# Autodesk Inventor assembly: BC-100000-Sup
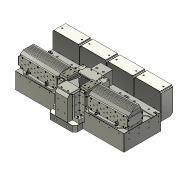
[picture p0: Inventor's stored thumbnail of the model, 180x180]
Saved by Autodesk Inventor 2016 (Build 200138000, 138)
## iProperties
Created: 2015-09-16
Part Number: BC-100000-Sup
Document SubType Name: Assembly
Designer: Reinaldo.Basílio
Mass: 567958 g
Surface Area: 49385.8 cm^2
Volume: 75452.4 cm^3
Density: 7.52737 g/cm^3
Author: Reinaldo.Basílio
## Documents named in this file (40)
- D:\ARQ\Basilio\LNLS-2\Anel\Dipolos\BC-3T\Dipolo 3T e 1T\Prototipo 1\Projeto Mecanico\BC-100000-Sup.iam
- D:\ARQ\Basilio\LNLS-2\Anel\Dipolos\BC-3T\Dipolo 3T e 1T\Prototipo 1\Projeto Mecanico\BC-100004.iam
- D:\ARQ\Basilio\LNLS-2\Anel\Dipolos\BC-3T\Dipolo 3T e 1T\Prototipo 1\Projeto Mecanico\BC-10005.ipt
- D:\ARQ\Basilio\LNLS-2\Anel\Dipolos\BC-3T\Dipolo 3T e 1T\Prototipo 1\Projeto Mecanico\BC-100005.iam
- D:\ARQ\Basilio\LNLS-2\Anel\Dipolos\BC-3T\Dipolo 3T e 1T\Prototipo 1\Projeto Mecanico\BC-10008.ipt
- D:\ARQ\Basilio\LNLS-2\Anel\Dipolos\BC-3T\Dipolo 3T e 1T\Prototipo 1\Projeto Mecanico\BC-10007.ipt
- D:\ARQ\Basilio\LNLS-2\Anel\Dipolos\BC-3T\Dipolo 3T e 1T\Prototipo 1\Projeto Mecanico\BC-10001.ipt
- D:\ARQ\Basilio\LNLS-2\Anel\Dipolos\BC-3T\Dipolo 3T e 1T\Prototipo 1\Projeto Mecanico\BC-10019-A.ipt
- D:\ARQ\Basilio\LNLS-2\Anel\Dipolos\BC-3T\Dipolo 3T e 1T\Prototipo 1\Projeto Mecanico\BC-10002.ipt
- D:\ARQ\Basilio\LNLS-2\Anel\Dipolos\BC-3T\Dipolo 3T e 1T\Prototipo 1\Projeto Mecanico\BC-10011.ipt
- D:\ARQ\Basilio\LNLS-2\Anel\Dipolos\BC-3T\Dipolo 3T e 1T\Prototipo 1\Projeto Mecanico\BC-10012.ipt
- D:\ARQ\Basilio\LNLS-2\Anel\Dipolos\BC-3T\Dipolo 3T e 1T\Prototipo 1\Projeto Mecanico\BC-10013.ipt
- D:\ARQ\Basilio\LNLS-2\Anel\Dipolos\BC-3T\Dipolo 3T e 1T\Prototipo 1\Projeto Mecanico\BC-10014.ipt
- D:\ARQ\Basilio\LNLS-2\Anel\Dipolos\BC-3T\Dipolo 3T e 1T\Prototipo 1\Projeto Mecanico\BC-10019-B.ipt
- D:\ARQ\Basilio\LNLS-2\Anel\Dipolos\BC-3T\Dipolo 3T e 1T\Prototipo 1\Projeto Mecanico\BC-10015.ipt
- D:\ARQ\Basilio\LNLS-2\Anel\Dipolos\BC-3T\Dipolo 3T e 1T\Prototipo 1\Projeto Mecanico\BC-10016.ipt
- D:\ARQ\Basilio\LNLS-2\Anel\Dipolos\BC-3T\Dipolo 3T e 1T\Prototipo 1\Projeto Mecanico\BC-10009.ipt
- D:\ARQ\Basilio\LNLS-2\Anel\Dipolos\BC-3T\Dipolo 3T e 1T\Prototipo 1\Projeto Mecanico\BC-100001-A-Sup.iam
- D:\ARQ\Basilio\LNLS-2\Anel\Dipolos\BC-3T\Dipolo 3T e 1T\Prototipo 1\Projeto Mecanico\BC-100001-B-Sup.iam
- D:\ARQ\Basilio\LNLS-2\Anel\Dipolos\BC-3T\Dipolo 3T e 1T\Prototipo 1\Projeto Mecanico\BC-10021.ipt
- D:\ARQ\Basilio\LNLS-2\Anel\Dipolos\BC-3T\Dipolo 3T e 1T\Prototipo 1\Projeto Mecanico\BC-10022.ipt
- D:\ARQ\Basilio\LNLS-2\Anel\Dipolos\BC-3T\Dipolo 3T e 1T\Prototipo 1\Projeto Mecanico\BC-10025.ipt
- D:\ARQ\Basilio\LNLS-2\Anel\Dipolos\BC-3T\Dipolo 3T e 1T\Prototipo 1\Projeto Mecanico\Parafusos\DIN 912 - M12x65.ipt
- D:\ARQ\Basilio\LNLS-2\Anel\Dipolos\BC-3T\Dipolo 3T e 1T\Prototipo 1\Projeto Mecanico\BC-10020.ipt
- D:\ARQ\Basilio\LNLS-2\Anel\Dipolos\BC-3T\Dipolo 3T e 1T\Prototipo 1\Projeto Mecanico\Parafusos\DIN 912 - M8x30.ipt
- D:\ARQ\Basilio\LNLS-2\Anel\Dipolos\BC-3T\Dipolo 3T e 1T\Prototipo 1\Projeto Mecanico\Parafusos\DIN 912 - M8x80.ipt
- D:\ARQ\Basilio\LNLS-2\Anel\Dipolos\BC-3T\Dipolo 3T e 1T\Prototipo 1\Projeto Mecanico\Parafusos\DIN 912 - M10x50.ipt
- D:\ARQ\Basilio\LNLS-2\Anel\Dipolos\BC-3T\Dipolo 3T e 1T\Prototipo 1\Projeto Mecanico\Parafusos\DIN 912 - M4x12.ipt
- D:\ARQ\Basilio\LNLS-2\Anel\Dipolos\BC-3T\Dipolo 3T e 1T\Prototipo 1\Projeto Mecanico\Parafusos\DIN 912 - M5x16.ipt
- D:\ARQ\Basilio\LNLS-2\Anel\Dipolos\BC-3T\Dipolo 3T e 1T\Prototipo 1\Projeto Mecanico\BC-10023.ipt
- D:\ARQ\Basilio\LNLS-2\Anel\Dipolos\BC-3T\Dipolo 3T e 1T\Prototipo 1\Projeto Mecanico\Parafusos\DIN 7991 - M5x12.ipt
- D:\ARQ\Basilio\LNLS-2\Anel\Dipolos\BC-3T\Dipolo 3T e 1T\Prototipo 1\Projeto Mecanico\Parafusos\DIN 125 - A 10,5.ipt
- D:\ARQ\Basilio\LNLS-2\Anel\Dipolos\BC-3T\Dipolo 3T e 1T\Prototipo 1\Projeto Mecanico\Parafusos\DIN 912 - M10x40.ipt
- D:\ARQ\Basilio\LNLS-2\Anel\Dipolos\BC-3T\Dipolo 3T e 1T\Prototipo 1\Projeto Mecanico\Parafusos\DIN 912 - M8x20.ipt
- D:\ARQ\Basilio\LNLS-2\Anel\Dipolos\BC-3T\Dipolo 3T e 1T\Prototipo 1\Projeto Mecanico\Parafusos\DIN 912 - M8x40.ipt
- D:\ARQ\Basilio\LNLS-2\Anel\Dipolos\BC-3T\Dipolo 3T e 1T\Prototipo 1\Projeto Mecanico\Parafusos\DIN 933 - M4x14.ipt
- D:\ARQ\Basilio\LNLS-2\Anel\Dipolos\BC-3T\Dipolo 3T e 1T\Prototipo 1\Projeto Mecanico\Parafusos\DIN 912 - M4x18.ipt
- D:\ARQ\Basilio\LNLS-2\Anel\Dipolos\BC-3T\Dipolo 3T e 1T\Prototipo 1\Projeto Mecanico\BC-10026.ipt
- D:\ARQ\Basilio\LNLS-2\Anel\Dipolos\BC-3T\Dipolo 3T e 1T\Prototipo 1\Projeto Mecanico\BC-10027.ipt
- D:\ARQ\Basilio\LNLS-2\Anel\Dipolos\BC-3T\Dipolo 3T e 1T\Prototipo 1\Projeto Mecanico\BC-100001\AIP\FEA\bjj5sjykh.fres
## Components (139 placed, 38 different names)
1. BC-10001:1 — Flush:41, Mate:39, Mate:48, Insert:3, Insert:6, Insert:7, Insert:8, Mate:54, Mate:55, Insert:13, Insert:15, Insert:16, Insert:22, Insert:23, Insert:24, Insert:25, Insert:26, Insert:27, Mate:57, Mate:62, Insert:30, Insert:31, Insert:36, Insert:37, Insert:38, Insert:39, Insert:40, Insert:41, Insert:42, Insert:43, Insert:44, Insert:45, Mate:67, Mate:70, Insert:61, Insert:62, Insert:71, Insert:72, Insert:73, Insert:74, Insert:75, Insert:76, Insert:77, Insert:78, Insert:167, Insert:168
2. BC-10002:1 — Flush:46, Mate:48, Insert:17, Insert:18, Insert:19, Insert:20, Insert:44, Insert:45, Flush:47, Insert:54, Insert:55, Insert:87, Insert:88
3. BC-100005:1 [sub-assembly] — Flush:28, Mate:67, Flush:47
4. BC-100004:1 [sub-assembly] — Mate:69, Flush:25, Mate:68, Mate:70
5. BC-10019-B:1 — Insert:13, Insert:14, Insert:131, Insert:132, Insert:133, Insert:134
6. BC-10019-A:2 — Mate:39, Mate:40, Mate:41, Insert:123, Insert:124, Insert:125, Insert:126
7. BC-10005:1 — Flush:25, Flush:28, Mate:22, Mate:24, Mate:28, Flush:33, Mate:29, Flush:34, Flush:41, Mate:40, Mate:41, Flush:46, Insert:14, Mate:68, Flush:48, Mate:71, Flush:49, Flush:51
8. BC-100004:2 [sub-assembly] — Mate:22, Flush:31, Flush:48
9. BC-100004:3 [sub-assembly] — Mate:24, Flush:50, Flush:51
10. BC-100005:2 [sub-assembly] — Flush:31, Flush:34, Mate:71, Flush:49, Flush:50
11. BC-10008:1 — Insert:28, Insert:29, Insert:30, Insert:31, Insert:46, Insert:47, Insert:48, Insert:49, Insert:93, Insert:94, Insert:95, Insert:96
12. BC-10007:1 — Insert:28, Insert:29
13. BC-100001-A-Sup:1 [sub-assembly] — Insert:3, Tangent:2, Mate:54
14. BC-100001-B-Sup:1 [sub-assembly] — Insert:6, Tangent:1, Mate:55
15. BC-10011:1 — Insert:8, Tangent:1, Insert:158
16. BC-10011:2 — Insert:7, Tangent:2, Insert:157
17. BC-10012:1 — Insert:15, Insert:16, Insert:149, Insert:150
18. BC-10014:1 — Insert:17, Insert:18, Insert:144, Insert:145, Insert:146, Insert:147, Insert:148
19. BC-10013:1 — Insert:19, Insert:20, Insert:139, Insert:140, Insert:141, Insert:142, Insert:143
20. BC-10012:2 — Insert:22, Insert:23, Mate:58, Insert:151, Insert:152
21. BC-10015:1 — Insert:24, Insert:25, Insert:89, Insert:90
22. BC-10015:2 — Insert:26, Insert:27, Insert:91, Insert:92
23. BC-10016:1 — Mate:57, Mate:58, Insert:48, Insert:49, Insert:107, Insert:108, Insert:153, Insert:154
24. BC-10016:2 — Mate:62, Insert:46, Insert:47, Insert:109, Insert:110, Insert:155, Insert:156
25. BC-10009:1 — Insert:36, Insert:37, Insert:63, Insert:64
26. BC-10009:2 — Insert:38, Insert:39, Insert:65, Insert:66
27. BC-10009:3 — Insert:40, Insert:41, Insert:67, Insert:68
28. BC-10009:4 — Insert:42, Insert:43, Insert:69, Insert:70
29. BC-10021:1 — Insert:54, Insert:55, Insert:56, Insert:57, Insert:59, Insert:60, Insert:99, Insert:100, Insert:101, Insert:102, Insert:103, Insert:104, Insert:105, Insert:106, Insert:111, Insert:112, Insert:113, Insert:114, Insert:169, Insert:170, Insert:171, Insert:172
30. BC-10022:1 — Insert:56, Insert:57, Insert:159, Insert:160, Insert:161, Insert:162
31. BC-10022:2 — Insert:59, Insert:60, Insert:163, Insert:164, Insert:165, Insert:166
32. BC-10025:1 — Insert:61, Insert:98
33. BC-10025:2 — Insert:62, Insert:97
34. DIN 912 - Parafuso Allen com cabeça (inox) M12x65:1 — Insert:63
35. DIN 912 - Parafuso Allen com cabeça (inox) M12x65:2 — Insert:64
36. DIN 912 - Parafuso Allen com cabeça (inox) M12x65:3 — Insert:65
37. DIN 912 - Parafuso Allen com cabeça (inox) M12x65:4 — Insert:66
38. DIN 912 - Parafuso Allen com cabeça (inox) M12x65:5 — Insert:67
39. DIN 912 - Parafuso Allen com cabeça (inox) M12x65:6 — Insert:68
40. DIN 912 - Parafuso Allen com cabeça (inox) M12x65:7 — Insert:69
41. DIN 912 - Parafuso Allen com cabeça (inox) M12x65:8 — Insert:70
42. BC-10020:1 — Insert:71, Insert:79
43. BC-10020:2 — Insert:73, Insert:80
44. BC-10020:3 — Insert:72, Insert:81
45. BC-10020:4 — Insert:74, Insert:82
46. BC-10020:5 — Insert:75, Insert:83
47. BC-10020:6 — Insert:77, Insert:84
48. BC-10020:7 — Insert:76, Insert:85
49. BC-10020:8 — Insert:78, Insert:86
50. DIN 912 - Parafuso Allen com cabeça (Inox) M8x30:1 — Insert:79
51. DIN 912 - Parafuso Allen com cabeça (Inox) M8x30:2 — Insert:80
52. DIN 912 - Parafuso Allen com cabeça (Inox) M8x30:3 — Insert:81
53. DIN 912 - Parafuso Allen com cabeça (Inox) M8x30:4 — Insert:82
54. DIN 912 - Parafuso Allen com cabeça (Inox) M8x30:5 — Insert:83
55. DIN 912 - Parafuso Allen com cabeça (Inox) M8x30:6 — Insert:84
56. DIN 912 - Parafuso Allen com cabeça (Inox) M8x30:7 — Insert:85
57. DIN 912 - Parafuso Allen com cabeça (Inox) M8x30:8 — Insert:86
58. DIN 912 - Parafuso Allen com cabeça (inox) M8x80:1 — Insert:87
59. DIN 912 - Parafuso Allen com cabeça (inox) M8x80:2 — Insert:88
60. DIN 912 - Parafuso Allen com cabeça (inox) M8x80:3 — Insert:89
61. DIN 912 - Parafuso Allen com cabeça (inox) M8x80:4 — Insert:90
62. DIN 912 - Parafuso Allen com cabeça (inox) M8x80:5 — Insert:91
63. DIN 912 - Parafuso Allen com cabeça (inox) M8x80:6 — Insert:92
64. DIN 912 - Parafuso Allen com cabeça (inox) M10x50:1 — Insert:93
65. DIN 912 - Parafuso Allen com cabeça (inox) M10x50:2 — Insert:94
66. DIN 912 - Parafuso Allen com cabeça (inox) M10x50:3 — Insert:96
67. DIN 912 - Parafuso Allen com cabeça (inox) M10x50:4 — Insert:95
68. DIN 912 - Aço Inox M4x12:1 — Insert:97
69. DIN 912 - Aço Inox M4x12:2 — Insert:98
70. DIN 912 - Aço Inox M5x16:1 — Insert:99
71. DIN 912 - Aço Inox M5x16:2 — Insert:100
72. DIN 912 - Aço Inox M5x16:3 — Insert:101
73. DIN 912 - Aço Inox M5x16:4 — Insert:102
74. DIN 912 - Aço Inox M5x16:5 — Insert:103
75. DIN 912 - Aço Inox M5x16:6 — Insert:104
76. DIN 912 - Aço Inox M5x16:7 — Insert:105
77. DIN 912 - Aço Inox M5x16:8 — Insert:106
78. BC-10023:1 — Insert:107, Insert:108, Insert:119, Insert:120, Insert:121, Insert:122
79. BC-10023:2 — Insert:109, Insert:110, Insert:115, Insert:116, Insert:117, Insert:118
80. DIN 7991 - Parafuso Allen com cabeça chata (inox) M5x12:1 — Insert:111
81. DIN 7991 - Parafuso Allen com cabeça chata (inox) M5x12:2 — Insert:112
82. DIN 7991 - Parafuso Allen com cabeça chata (inox) M5x12:3 — Insert:114
83. DIN 7991 - Parafuso Allen com cabeça chata (inox) M5x12:4 — Insert:113
84. DIN 7991 - Parafuso Allen com cabeça chata (inox) M5x12:5 — Insert:116
85. DIN 7991 - Parafuso Allen com cabeça chata (inox) M5x12:6 — Insert:115
86. DIN 7991 - Parafuso Allen com cabeça chata (inox) M5x12:7 — Insert:118
87. DIN 7991 - Parafuso Allen com cabeça chata (inox) M5x12:8 — Insert:117
88. DIN 7991 - Parafuso Allen com cabeça chata (inox) M5x12:9 — Insert:119
89. DIN 7991 - Parafuso Allen com cabeça chata (inox) M5x12:10 — Insert:120
90. DIN 7991 - Parafuso Allen com cabeça chata (inox) M5x12:11 — Insert:121
91. DIN 7991 - Parafuso Allen com cabeça chata (inox) M5x12:12 — Insert:122
92. DIN 125 A - Aço Inox 316 A 10,5:1 — Insert:123, Insert:127
93. DIN 125 A - Aço Inox 316 A 10,5:2 — Insert:124, Insert:128
94. DIN 125 A - Aço Inox 316 A 10,5:3 — Insert:125, Insert:129
95. DIN 125 A - Aço Inox 316 A 10,5:4 — Insert:126, Insert:130
96. DIN 912 - Parafuso Allen com cabeça (inox) M10x40:1 — Insert:127
97. DIN 912 - Parafuso Allen com cabeça (inox) M10x40:2 — Insert:128
98. DIN 912 - Parafuso Allen com cabeça (inox) M10x40:3 — Insert:129
99. DIN 912 - Parafuso Allen com cabeça (inox) M10x40:4 — Insert:130
100. DIN 125 A - Aço Inox 316 A 10,5:5 — Insert:131, Insert:135
101. DIN 125 A - Aço Inox 316 A 10,5:6 — Insert:132, Insert:136
102. DIN 125 A - Aço Inox 316 A 10,5:7 — Insert:133, Insert:137
103. DIN 125 A - Aço Inox 316 A 10,5:8 — Insert:134, Insert:138
104. DIN 912 - Parafuso Allen com cabeça (inox) M10x40:5 — Insert:135
105. DIN 912 - Parafuso Allen com cabeça (inox) M10x40:6 — Insert:136
106. DIN 912 - Parafuso Allen com cabeça (inox) M10x40:7 — Insert:137
107. DIN 912 - Parafuso Allen com cabeça (inox) M10x40:8 — Insert:138
108. DIN 912 - Parafuso Allen com cabeça (Inox) M8x20:1 — Insert:139
109. DIN 912 - Parafuso Allen com cabeça (Inox) M8x20:2 — Insert:140
110. DIN 912 - Parafuso Allen com cabeça (Inox) M8x20:3 — Insert:141
111. DIN 912 - Parafuso Allen com cabeça (Inox) M8x20:4 — Insert:142
112. DIN 912 - Parafuso Allen com cabeça (Inox) M8x20:5 — Insert:143
113. DIN 912 - Parafuso Allen com cabeça (Inox) M8x20:6 — Insert:144
114. DIN 912 - Parafuso Allen com cabeça (Inox) M8x20:7 — Insert:145
115. DIN 912 - Parafuso Allen com cabeça (Inox) M8x20:8 — Insert:146
116. DIN 912 - Parafuso Allen com cabeça (Inox) M8x20:9 — Insert:147
117. DIN 912 - Parafuso Allen com cabeça (Inox) M8x20:10 — Insert:148
118. DIN 912 - Parafuso Allen com cabeça (Inox) M8x30:9 — Insert:149
119. DIN 912 - Parafuso Allen com cabeça (Inox) M8x30:10 — Insert:150
120. DIN 912 - Parafuso Allen com cabeça (Inox) M8x30:11 — Insert:151
121. DIN 912 - Parafuso Allen com cabeça (Inox) M8x30:12 — Insert:152
122. DIN 912 - Parafuso Allen com cabeça (Inox) M8x40:1 — Insert:153
123. DIN 912 - Parafuso Allen com cabeça (Inox) M8x40:2 — Insert:154
124. DIN 912 - Parafuso Allen com cabeça (Inox) M8x40:3 — Insert:155
125. DIN 912 - Parafuso Allen com cabeça (Inox) M8x40:4 — Insert:156
126. DIN 933 - Parafuso sextavado com rosca total  M4x20:1 — Insert:157
127. DIN 933 - Parafuso sextavado com rosca total  M4x20:2 — Insert:158
128. DIN 912 - Aço Inox M4x18:1 — Insert:159
129. DIN 912 - Aço Inox M4x18:2 — Insert:160
130. DIN 912 - Aço Inox M4x18:3 — Insert:161
131. DIN 912 - Aço Inox M4x18:4 — Insert:162
132. DIN 912 - Aço Inox M4x18:5 — Insert:164
133. DIN 912 - Aço Inox M4x18:6 — Insert:163
134. DIN 912 - Aço Inox M4x18:7 — Insert:165
135. DIN 912 - Aço Inox M4x18:8 — Insert:166
136. BC-10026:1 — Insert:167
137. BC-10026:2 — Insert:168
138. BC-10027:1 — Insert:169, Insert:170
139. BC-10027:2 — Insert:171, Insert:172
## Relationships (186: Insert 154, Mate 18, Flush 12, Tangent 2)
- Mate:69: BC-100004:1
- Flush:25: BC-100004:1 ↔ BC-10005:1
- Flush:28: BC-100005:1 ↔ BC-10005:1
- Mate:22: BC-10005:1 ↔ BC-100004:2
- Mate:24: BC-10005:1 ↔ BC-100004:3
- Flush:31: BC-100004:2 ↔ BC-100005:2
- Mate:28: BC-10005:1
- Flush:33: BC-10005:1
- Mate:29: BC-10005:1
- Flush:34 (-30 mm): BC-10005:1 ↔ BC-100005:2
- Flush:41: BC-10001:1 ↔ BC-10005:1
- Mate:39: BC-10001:1 ↔ BC-10019-A:2
- Mate:40: BC-10019-A:2 ↔ BC-10005:1
- Mate:41: BC-10019-A:2 ↔ BC-10005:1
- Flush:46: BC-10002:1 ↔ BC-10005:1
- Mate:48: BC-10001:1 ↔ BC-10002:1
- Insert:3: BC-10001:1 ↔ BC-100001-A-Sup:1
- Insert:6: BC-10001:1 ↔ BC-100001-B-Sup:1
- Insert:7: BC-10001:1 ↔ BC-10011:2
- Insert:8: BC-10001:1 ↔ BC-10011:1
- Tangent:1: BC-100001-B-Sup:1 ↔ BC-10011:1
- Tangent:2: BC-100001-A-Sup:1 ↔ BC-10011:2
- Mate:54: BC-10001:1 ↔ BC-100001-A-Sup:1
- Mate:55: BC-10001:1 ↔ BC-100001-B-Sup:1
- Insert:13: BC-10001:1 ↔ BC-10019-B:1
- Insert:14: BC-10019-B:1 ↔ BC-10005:1
- Insert:15: BC-10001:1 ↔ BC-10012:1
- Insert:16: BC-10001:1 ↔ BC-10012:1
- Insert:17: BC-10002:1 ↔ BC-10014:1
- Insert:18: BC-10002:1 ↔ BC-10014:1
- Insert:19: BC-10002:1 ↔ BC-10013:1
- Insert:20: BC-10002:1 ↔ BC-10013:1
- Insert:22: BC-10001:1 ↔ BC-10012:2
- Insert:23: BC-10001:1 ↔ BC-10012:2
- Insert:24: BC-10001:1 ↔ BC-10015:1
- Insert:25: BC-10001:1 ↔ BC-10015:1
- Insert:26: BC-10001:1 ↔ BC-10015:2
- Insert:27: BC-10001:1 ↔ BC-10015:2
- Mate:57: BC-10001:1 ↔ BC-10016:1
- Mate:58: BC-10012:2 ↔ BC-10016:1
- Mate:62: BC-10001:1 ↔ BC-10016:2
- Insert:28: BC-10008:1 ↔ BC-10007:1
- Insert:29: BC-10008:1 ↔ BC-10007:1
- Insert:30: BC-10001:1 ↔ BC-10008:1
- Insert:31: BC-10001:1 ↔ BC-10008:1
- Insert:36: BC-10001:1 ↔ BC-10009:1
- Insert:37: BC-10001:1 ↔ BC-10009:1
- Insert:38: BC-10001:1 ↔ BC-10009:2
- Insert:39: BC-10001:1 ↔ BC-10009:2
- Insert:40: BC-10001:1 ↔ BC-10009:3
- Insert:41: BC-10001:1 ↔ BC-10009:3
- Insert:42: BC-10001:1 ↔ BC-10009:4
- Insert:43: BC-10001:1 ↔ BC-10009:4
- Insert:44: BC-10001:1 ↔ BC-10002:1
- Insert:45: BC-10001:1 ↔ BC-10002:1
- Mate:67: BC-10001:1 ↔ BC-100005:1
- Flush:47: BC-10002:1 ↔ BC-100005:1
- Mate:68: BC-100004:1 ↔ BC-10005:1
- Flush:48: BC-10005:1 ↔ BC-100004:2
- Mate:70: BC-10001:1 ↔ BC-100004:1
- Mate:71: BC-10005:1 ↔ BC-100005:2
- Flush:49: BC-10005:1 ↔ BC-100005:2
- Flush:50: BC-100004:3 ↔ BC-100005:2
- Flush:51: BC-10005:1 ↔ BC-100004:3
- Insert:46: BC-10008:1 ↔ BC-10016:2
- Insert:47: BC-10008:1 ↔ BC-10016:2
- Insert:48: BC-10008:1 ↔ BC-10016:1
- Insert:49: BC-10008:1 ↔ BC-10016:1
- Insert:54: BC-10002:1 ↔ BC-10021:1
- Insert:55: BC-10002:1 ↔ BC-10021:1
- Insert:56 (2.6 mm): BC-10021:1 ↔ BC-10022:1
- Insert:57 (2.6 mm): BC-10021:1 ↔ BC-10022:1
- Insert:59 (2.6 mm): BC-10021:1 ↔ BC-10022:2
- Insert:60 (2.6 mm): BC-10021:1 ↔ BC-10022:2
- Insert:61: BC-10001:1 ↔ BC-10025:1
- Insert:62: BC-10001:1 ↔ BC-10025:2
- Insert:63: BC-10009:1 ↔ DIN 912 - Parafuso Allen com cabeça (inox) M12x65:1
- Insert:64: BC-10009:1 ↔ DIN 912 - Parafuso Allen com cabeça (inox) M12x65:2
- Insert:65: BC-10009:2 ↔ DIN 912 - Parafuso Allen com cabeça (inox) M12x65:3
- Insert:66: BC-10009:2 ↔ DIN 912 - Parafuso Allen com cabeça (inox) M12x65:4
- Insert:67: BC-10009:3 ↔ DIN 912 - Parafuso Allen com cabeça (inox) M12x65:5
- Insert:68: BC-10009:3 ↔ DIN 912 - Parafuso Allen com cabeça (inox) M12x65:6
- Insert:69: BC-10009:4 ↔ DIN 912 - Parafuso Allen com cabeça (inox) M12x65:7
- Insert:70: BC-10009:4 ↔ DIN 912 - Parafuso Allen com cabeça (inox) M12x65:8
- Insert:71 (12.5 mm): BC-10001:1 ↔ BC-10020:1
- Insert:72 (12.5 mm): BC-10001:1 ↔ BC-10020:3
- Insert:73 (12.5 mm): BC-10001:1 ↔ BC-10020:2
- Insert:74 (12.5 mm): BC-10001:1 ↔ BC-10020:4
- Insert:75 (12.5 mm): BC-10001:1 ↔ BC-10020:5
- Insert:76 (12.5 mm): BC-10001:1 ↔ BC-10020:7
- Insert:77 (12.5 mm): BC-10001:1 ↔ BC-10020:6
- Insert:78 (12.5 mm): BC-10001:1 ↔ BC-10020:8
- Insert:79: BC-10020:1 ↔ DIN 912 - Parafuso Allen com cabeça (Inox) M8x30:1
- Insert:80: BC-10020:2 ↔ DIN 912 - Parafuso Allen com cabeça (Inox) M8x30:2
- Insert:81: BC-10020:3 ↔ DIN 912 - Parafuso Allen com cabeça (Inox) M8x30:3
- Insert:82: BC-10020:4 ↔ DIN 912 - Parafuso Allen com cabeça (Inox) M8x30:4
- Insert:83: BC-10020:5 ↔ DIN 912 - Parafuso Allen com cabeça (Inox) M8x30:5
- Insert:84: BC-10020:6 ↔ DIN 912 - Parafuso Allen com cabeça (Inox) M8x30:6
- Insert:85: BC-10020:7 ↔ DIN 912 - Parafuso Allen com cabeça (Inox) M8x30:7
- Insert:86: BC-10020:8 ↔ DIN 912 - Parafuso Allen com cabeça (Inox) M8x30:8
- Insert:87: BC-10002:1 ↔ DIN 912 - Parafuso Allen com cabeça (inox) M8x80:1
- Insert:88: BC-10002:1 ↔ DIN 912 - Parafuso Allen com cabeça (inox) M8x80:2
- Insert:89: BC-10015:1 ↔ DIN 912 - Parafuso Allen com cabeça (inox) M8x80:3
- Insert:90: BC-10015:1 ↔ DIN 912 - Parafuso Allen com cabeça (inox) M8x80:4
- Insert:91: BC-10015:2 ↔ DIN 912 - Parafuso Allen com cabeça (inox) M8x80:5
- Insert:92: BC-10015:2 ↔ DIN 912 - Parafuso Allen com cabeça (inox) M8x80:6
- Insert:93: BC-10008:1 ↔ DIN 912 - Parafuso Allen com cabeça (inox) M10x50:1
- Insert:94: BC-10008:1 ↔ DIN 912 - Parafuso Allen com cabeça (inox) M10x50:2
- Insert:95: BC-10008:1 ↔ DIN 912 - Parafuso Allen com cabeça (inox) M10x50:4
- Insert:96: BC-10008:1 ↔ DIN 912 - Parafuso Allen com cabeça (inox) M10x50:3
- Insert:97: BC-10025:2 ↔ DIN 912 - Aço Inox M4x12:1
- Insert:98: BC-10025:1 ↔ DIN 912 - Aço Inox M4x12:2
- Insert:99: BC-10021:1 ↔ DIN 912 - Aço Inox M5x16:1
- Insert:100: BC-10021:1 ↔ DIN 912 - Aço Inox M5x16:2
- Insert:101: BC-10021:1 ↔ DIN 912 - Aço Inox M5x16:3
- Insert:102: BC-10021:1 ↔ DIN 912 - Aço Inox M5x16:4
- Insert:103: BC-10021:1 ↔ DIN 912 - Aço Inox M5x16:5
- Insert:104: BC-10021:1 ↔ DIN 912 - Aço Inox M5x16:6
- Insert:105: BC-10021:1 ↔ DIN 912 - Aço Inox M5x16:7
- Insert:106: BC-10021:1 ↔ DIN 912 - Aço Inox M5x16:8
- Insert:107: BC-10016:1 ↔ BC-10023:1
- Insert:108: BC-10016:1 ↔ BC-10023:1
- Insert:109: BC-10016:2 ↔ BC-10023:2
- Insert:110: BC-10016:2 ↔ BC-10023:2
- Insert:111: BC-10021:1 ↔ DIN 7991 - Parafuso Allen com cabeça chata (inox) M5x12:1
- Insert:112: BC-10021:1 ↔ DIN 7991 - Parafuso Allen com cabeça chata (inox) M5x12:2
- Insert:113: BC-10021:1 ↔ DIN 7991 - Parafuso Allen com cabeça chata (inox) M5x12:4
- Insert:114: BC-10021:1 ↔ DIN 7991 - Parafuso Allen com cabeça chata (inox) M5x12:3
- Insert:115: BC-10023:2 ↔ DIN 7991 - Parafuso Allen com cabeça chata (inox) M5x12:6
- Insert:116: BC-10023:2 ↔ DIN 7991 - Parafuso Allen com cabeça chata (inox) M5x12:5
- Insert:117: BC-10023:2 ↔ DIN 7991 - Parafuso Allen com cabeça chata (inox) M5x12:8
- Insert:118: BC-10023:2 ↔ DIN 7991 - Parafuso Allen com cabeça chata (inox) M5x12:7
- Insert:119: BC-10023:1 ↔ DIN 7991 - Parafuso Allen com cabeça chata (inox) M5x12:9
- Insert:120: BC-10023:1 ↔ DIN 7991 - Parafuso Allen com cabeça chata (inox) M5x12:10
- Insert:121: BC-10023:1 ↔ DIN 7991 - Parafuso Allen com cabeça chata (inox) M5x12:11
- Insert:122: BC-10023:1 ↔ DIN 7991 - Parafuso Allen com cabeça chata (inox) M5x12:12
- Insert:123: BC-10019-A:2 ↔ DIN 125 A - Aço Inox 316 A 10,5:1
- Insert:124: BC-10019-A:2 ↔ DIN 125 A - Aço Inox 316 A 10,5:2
- Insert:125: BC-10019-A:2 ↔ DIN 125 A - Aço Inox 316 A 10,5:3
- Insert:126: BC-10019-A:2 ↔ DIN 125 A - Aço Inox 316 A 10,5:4
- Insert:127: DIN 125 A - Aço Inox 316 A 10,5:1 ↔ DIN 912 - Parafuso Allen com cabeça (inox) M10x40:1
- Insert:128: DIN 125 A - Aço Inox 316 A 10,5:2 ↔ DIN 912 - Parafuso Allen com cabeça (inox) M10x40:2
- Insert:129: DIN 125 A - Aço Inox 316 A 10,5:3 ↔ DIN 912 - Parafuso Allen com cabeça (inox) M10x40:3
- Insert:130: DIN 125 A - Aço Inox 316 A 10,5:4 ↔ DIN 912 - Parafuso Allen com cabeça (inox) M10x40:4
- Insert:131: BC-10019-B:1 ↔ DIN 125 A - Aço Inox 316 A 10,5:5
- Insert:132: BC-10019-B:1 ↔ DIN 125 A - Aço Inox 316 A 10,5:6
- Insert:133: BC-10019-B:1 ↔ DIN 125 A - Aço Inox 316 A 10,5:7
- Insert:134: BC-10019-B:1 ↔ DIN 125 A - Aço Inox 316 A 10,5:8
- Insert:135: DIN 125 A - Aço Inox 316 A 10,5:5 ↔ DIN 912 - Parafuso Allen com cabeça (inox) M10x40:5
- Insert:136: DIN 125 A - Aço Inox 316 A 10,5:6 ↔ DIN 912 - Parafuso Allen com cabeça (inox) M10x40:6
- Insert:137: DIN 125 A - Aço Inox 316 A 10,5:7 ↔ DIN 912 - Parafuso Allen com cabeça (inox) M10x40:7
- Insert:138: DIN 125 A - Aço Inox 316 A 10,5:8 ↔ DIN 912 - Parafuso Allen com cabeça (inox) M10x40:8
- Insert:139: BC-10013:1 ↔ DIN 912 - Parafuso Allen com cabeça (Inox) M8x20:1
- Insert:140: BC-10013:1 ↔ DIN 912 - Parafuso Allen com cabeça (Inox) M8x20:2
- Insert:141: BC-10013:1 ↔ DIN 912 - Parafuso Allen com cabeça (Inox) M8x20:3
- Insert:142: BC-10013:1 ↔ DIN 912 - Parafuso Allen com cabeça (Inox) M8x20:4
- Insert:143: BC-10013:1 ↔ DIN 912 - Parafuso Allen com cabeça (Inox) M8x20:5
- Insert:144: BC-10014:1 ↔ DIN 912 - Parafuso Allen com cabeça (Inox) M8x20:6
- Insert:145: BC-10014:1 ↔ DIN 912 - Parafuso Allen com cabeça (Inox) M8x20:7
- Insert:146: BC-10014:1 ↔ DIN 912 - Parafuso Allen com cabeça (Inox) M8x20:8
- Insert:147: BC-10014:1 ↔ DIN 912 - Parafuso Allen com cabeça (Inox) M8x20:9
- Insert:148: BC-10014:1 ↔ DIN 912 - Parafuso Allen com cabeça (Inox) M8x20:10
- Insert:149: BC-10012:1 ↔ DIN 912 - Parafuso Allen com cabeça (Inox) M8x30:9
- Insert:150: BC-10012:1 ↔ DIN 912 - Parafuso Allen com cabeça (Inox) M8x30:10
- Insert:151: BC-10012:2 ↔ DIN 912 - Parafuso Allen com cabeça (Inox) M8x30:11
- Insert:152: BC-10012:2 ↔ DIN 912 - Parafuso Allen com cabeça (Inox) M8x30:12
- Insert:153: BC-10016:1 ↔ DIN 912 - Parafuso Allen com cabeça (Inox) M8x40:1
- Insert:154: BC-10016:1 ↔ DIN 912 - Parafuso Allen com cabeça (Inox) M8x40:2
- Insert:155: BC-10016:2 ↔ DIN 912 - Parafuso Allen com cabeça (Inox) M8x40:3
- Insert:156: BC-10016:2 ↔ DIN 912 - Parafuso Allen com cabeça (Inox) M8x40:4
- Insert:157: BC-10011:2 ↔ DIN 933 - Parafuso sextavado com rosca total  M4x20:1
- Insert:158: BC-10011:1 ↔ DIN 933 - Parafuso sextavado com rosca total  M4x20:2
- Insert:159: BC-10022:1 ↔ DIN 912 - Aço Inox M4x18:1
- Insert:160: BC-10022:1 ↔ DIN 912 - Aço Inox M4x18:2
- Insert:161: BC-10022:1 ↔ DIN 912 - Aço Inox M4x18:3
- Insert:162: BC-10022:1 ↔ DIN 912 - Aço Inox M4x18:4
- Insert:163: BC-10022:2 ↔ DIN 912 - Aço Inox M4x18:6
- Insert:164: BC-10022:2 ↔ DIN 912 - Aço Inox M4x18:5
- Insert:165: BC-10022:2 ↔ DIN 912 - Aço Inox M4x18:7
- Insert:166: BC-10022:2 ↔ DIN 912 - Aço Inox M4x18:8
- Insert:167: BC-10001:1 ↔ BC-10026:1
- Insert:168: BC-10001:1 ↔ BC-10026:2
- Insert:169: BC-10021:1 ↔ BC-10027:1
- Insert:170: BC-10021:1 ↔ BC-10027:1
- Insert:171: BC-10021:1 ↔ BC-10027:2
- Insert:172: BC-10021:1 ↔ BC-10027:2
